# Autodesk Inventor assembly: rightHalfOfFrameV03
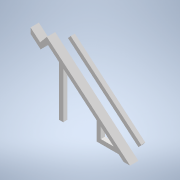
[picture p0: Inventor's stored thumbnail of the model, 180x180]
Saved by Autodesk Inventor 2020.2 (Build 242310000, 310)
## iProperties
Created: 2020-02-22
Part Number: rightHalfOfFrameV03
Document SubType Name: Assembly
Designer: robst
Author: robst
## Documents named in this file (4)
- C:\git\CAD-Development\robSteele\2020LongRobotBase\rightHalfOfFrameV03.iam
- C:\git\CAD-Development\robSteele\2020LongRobotBase\newFrame1x2piecsV03.ipt
- C:\git\CAD-Development\robSteele\2020LongRobotBase\newFrame1x1V03.ipt
- C:\git\CAD-Development\robSteele\2020LongRobotBase\newPullyV03.ipt
## Components (3 placed, 3 different names)
1. newFrame1x1V03:1 — Mate:1, Flush:1, Flush:2
2. newFrame1x2piecsV03:1 — Mate:1, Flush:1, Flush:2, Flush:3, Mate:2, Flush:4
3. newPullyV03:1 — Flush:3, Mate:2, Flush:4
## Relationships (6: Flush 4, Mate 2)
- Mate:1: newFrame1x1V03:1 ↔ newFrame1x2piecsV03:1
- Flush:1: newFrame1x1V03:1 ↔ newFrame1x2piecsV03:1
- Flush:2: newFrame1x1V03:1 ↔ newFrame1x2piecsV03:1
- Flush:3 (63.5 mm): newFrame1x2piecsV03:1 ↔ newPullyV03:1
- Mate:2 (127 mm): newFrame1x2piecsV03:1 ↔ newPullyV03:1
- Flush:4: newFrame1x2piecsV03:1 ↔ newPullyV03:1
